# Autodesk Inventor assembly: 84T HS Gear With Insert.ipt
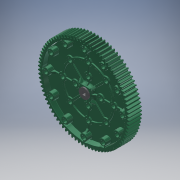
[picture p0: Inventor's stored thumbnail of the model, 180x180]
Saved by Autodesk Inventor 2019 (Build 230136000, 136)
## iProperties
Created: 2019-11-17
Part Number: 84T HS Gear With Insert.ipt
Document SubType Name: Assembly
Designer: karlv
Author: karlv
## Documents named in this file (3)
- C:\Users\karlv\Documents\VEX\Karl CAD Lib\KarlCADLib\Gears\HS\84T HS Gear With Insert.ipt.iam
- C:\Users\karlv\Documents\VEX\Karl CAD Lib\KarlCADLib\Gears\HS\84T HS Gear.ipt
- C:\Users\karlv\Documents\VEX\Karl CAD Lib\KarlCADLib\Gears\Inserts\Locked Metal Inserts.ipt
## Components (3 placed, 2 different names)
1. 84T HS Gear:1 — Mate:1, Mate:2, Mate:3, Mate:4, Mate:5, Mate:6
2. Locked Metal Inserts:1 — Mate:1, Mate:2, Mate:3
3. Locked Metal Inserts:2 — Mate:4, Mate:5, Mate:6
## Relationships (6: Mate 6)
- Mate:1: 84T HS Gear:1 ↔ Locked Metal Inserts:1
- Mate:2: 84T HS Gear:1 ↔ Locked Metal Inserts:1
- Mate:3: 84T HS Gear:1 ↔ Locked Metal Inserts:1
- Mate:4: 84T HS Gear:1 ↔ Locked Metal Inserts:2
- Mate:5: 84T HS Gear:1 ↔ Locked Metal Inserts:2
- Mate:6: 84T HS Gear:1 ↔ Locked Metal Inserts:2
